# Autodesk Inventor assembly: NoSpace2.0
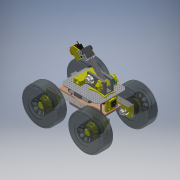
[picture p0: Inventor's stored thumbnail of the model, 180x180]
Saved by Autodesk Inventor 2019.1 (Build 231200000, 200)
## iProperties
Created: 2018-10-15
Part Number: NoSpace2.0
Material: Типовые
Document SubType Name: Assembly
Designer: Олег
Author: Олег
## Documents named in this file (34)
- C:\Users\Олег\OneDrive\Общая\NoSpace 2.0\NoSpace2.0.iam
- C:\Users\Олег\OneDrive\Общая\NoSpace 2.0\Основная пластина платформы.ipt
- C:\Users\Олег\OneDrive\Общая\NoSpace 2.0\Линейка.ipt
- C:\Users\Олег\OneDrive\Общая\NoSpace 2.0\Мотор-колесо\Мотор-колесо.iam
- C:\Users\Олег\OneDrive\Общая\NoSpace 2.0\Стойка между первым и вторым этажом.ipt
- C:\Users\Олег\OneDrive\Общая\NoSpace 2.0\Перфорированная пластина второго этажа.ipt
- C:\Users\Олег\OneDrive\Общая\NoSpace 2.0\Манипулятор\Поворотный узел манипулятора\Поворотный узел манипулятора.iam
- C:\Users\Олег\OneDrive\Общая\NoSpace 2.0\Крепление платы раздачи питания.ipt
- C:\Users\Олег\OneDrive\Общая\NoSpace 2.0\Держатель драйвера.ipt
- C:\Users\Олег\OneDrive\Общая\NoSpace 2.0\Малина.ipt
- C:\Users\Олег\OneDrive\Общая\NoSpace 2.0\стойка для платы 10мм.ipt
- C:\Users\Олег\OneDrive\Общая\NoSpace 2.0\bullet корпус.ipt
- C:\Users\Олег\OneDrive\Общая\NoSpace 2.0\bullet крышка.ipt
- C:\Users\Олег\OneDrive\Общая\NoSpace 2.0\Крепление АКБ.ipt
- C:\Users\Олег\OneDrive\Общая\NoSpace 2.0\Камера\Камера raspberry pi.ipt
- C:\Users\Олег\OneDrive\Общая\NoSpace 2.0\Камера\Основа камеры.ipt
- C:\Users\Олег\OneDrive\Общая\NoSpace 2.0\Камера\Поворотная платформа камеры.ipt
- C:\Users\Олег\OneDrive\Общая\NoSpace 2.0\Камера\Проставка между камерой и поворотной платформой.ipt
- C:\Users\Олег\OneDrive\Общая\NoSpace 2.0\Камера\Фиксатор подшипнкиа камеры.ipt
- C:\Users\Олег\OneDrive\Общая\NoSpace 2.0\Камера\Servo-MG90S.ipt
- C:\Users\Олег\OneDrive\Общая\NoSpace 2.0\Камера\Подшипник 3x10x4.ipt
- C:\Users\Олег\OneDrive\Общая\NoSpace 2.0\Манипулятор\Блок подъёма первога звена\Основная часть подъемного механизма первого звена.iam
- C:\Users\Олег\OneDrive\Общая\NoSpace 2.0\Манипулятор\Блок подъёма первога звена\Ось подъёмного блока первого звена.ipt
- C:\Users\Олег\OneDrive\Общая\NoSpace 2.0\Манипулятор\Блок подъёма первога звена\Узел потенциометра.iam
- C:\Users\Олег\OneDrive\Общая\NoSpace 2.0\Манипулятор\Блок подъёма первога звена\Шкив.iam
- C:\Users\Олег\OneDrive\Общая\NoSpace 2.0\Мотор-колесо\Мотор\Мотор.iam
- C:\Users\Олег\OneDrive\Общая\NoSpace 2.0\Манипулятор\Блок подъёма первога звена\Съёмное крепление мотора 37мм.ipt
- C:\Users\Олег\OneDrive\Общая\NoSpace 2.0\Манипулятор\Блок подъёма первога звена\Переходник от первого звена к оси.ipt
- C:\Users\Олег\OneDrive\Общая\NoSpace 2.0\Манипулятор\Блок подъёма первога звена\Шкив.ipt
- C:\Users\Олег\OneDrive\Общая\NoSpace 2.0\Манипулятор\Удлинение звена.ipt
- C:\Users\Олег\OneDrive\Общая\NoSpace 2.0\Манипулятор\Servoarm 1 RDS3115mg.ipt
- C:\Users\Олег\OneDrive\Общая\NoSpace 2.0\Манипулятор\RDS3115 MG.ipt
- C:\Users\Олег\OneDrive\Общая\NoSpace 2.0\Манипулятор\Поворотный узел схвата\Поворотный узел схвата.iam
- C:\Users\Олег\OneDrive\Общая\NoSpace 2.0\Манипулятор\Крепление схвата.ipt
## Components (47 placed, 33 different names)
1. Основная пластина платформы:1 — Совмещение:1, Совмещение:2, Совмещение:3, Совмещение:4, Совмещение:5, Совмещение:6, Совмещение:19, Совмещение:20, Совмещение:21, Совмещение:22, Совмещение:23, Совмещение:24, Совмещение:25, Совмещение:26, Совмещение:33, Совмещение:34, Совмещение:35, Совмещение:36, Совмещение:37, Совмещение:38, Совмещение:39, Заподлицо:1, Совмещение:41, Совмещение:42, Совмещение:43, Совмещение:44, Совмещение:45, Совмещение:46, Совмещение:48
2. Линейка:1 — Совмещение:4, Совмещение:5, Совмещение:6, Совмещение:13, Совмещение:14, Совмещение:15, Совмещение:16, Совмещение:17, Совмещение:18
3. Линейка:2 — Совмещение:1, Совмещение:2, Совмещение:3, Совмещение:7, Совмещение:8, Совмещение:9, Совмещение:10, Совмещение:11, Совмещение:12
4. Мотор-колесо:1 [sub-assembly] — Совмещение:10, Совмещение:11, Совмещение:12
5. Мотор-колесо:2 [sub-assembly] — Совмещение:13, Совмещение:14, Совмещение:15
6. Мотор-колесо:3 [sub-assembly] — Совмещение:16, Совмещение:17, Совмещение:18
7. Мотор-колесо:4 [sub-assembly] — Совмещение:7, Совмещение:8, Совмещение:9
8. Стойка между первым и вторым этажом:1 — Совмещение:25, Совмещение:26, Совмещение:27
9. Стойка между первым и вторым этажом:2 — Совмещение:23, Совмещение:24, Совмещение:28, Совмещение:29
10. Стойка между первым и вторым этажом:3 — Совмещение:21, Совмещение:22
11. Стойка между первым и вторым этажом:4 — Совмещение:19, Совмещение:20
12. Перфорированная пластина второго этажа:1 — Совмещение:27, Совмещение:28, Совмещение:29, Совмещение:30, Совмещение:31, Совмещение:32, Совмещение:52, Совмещение:53, Совмещение:54, Совмещение:56, Совмещение:57, Совмещение:58, Совмещение:62, Угол:1, Совмещение:63, Совмещение:64
13. Поворотный узел манипулятора:1 [sub-assembly] — Совмещение:30, Совмещение:31, Совмещение:32, Совмещение:77, Совмещение:78
14. Крепление платы раздачи питания:1 — Совмещение:33, Совмещение:34, Совмещение:35
15. Держатель драйвера:1 — Совмещение:36, Совмещение:37, Совмещение:38, Совмещение:40
16. Малина:1 — Совмещение:39, Совмещение:40, Заподлицо:1, Совмещение:47
17. стойка для платы 10мм:1 — Совмещение:41, Совмещение:42
18. стойка для платы 10мм:2 — Совмещение:44, Совмещение:47
19. стойка для платы 10мм:3 — Совмещение:43, Совмещение:48
20. стойка для платы 10мм:4 — Совмещение:45, Совмещение:46
21. bullet корпус:1 — Заподлицо:2, Заподлицо:3, Совмещение:55, Совмещение:56, Совмещение:57, Совмещение:58
22. bullet крышка:1 — Заподлицо:2, Заподлицо:3, Совмещение:55
23. Крепление АКБ:1 — Совмещение:49, Совмещение:50, Совмещение:51, Совмещение:52, Совмещение:54
24. Крепление АКБ:2 — Совмещение:49, Совмещение:50, Совмещение:51, Совмещение:53
25. Камера raspberry pi:1 — Совмещение:74, Совмещение:75, Совмещение:76
26. Основа камеры:1 — Совмещение:59, Совмещение:60, Совмещение:61, Совмещение:62, Угол:1, Совмещение:63, Совмещение:64, Совмещение:72, Совмещение:73
27. Поворотная платформа камеры:1 — Совмещение:67, Совмещение:68, Совмещение:69, Совмещение:70, Заподлицо:4, Заподлицо:5, Совмещение:72
28. Проставка между камерой и поворотной платформой:1 — Совмещение:70, Заподлицо:4, Заподлицо:5, Совмещение:74, Совмещение:75, Совмещение:76
29. Фиксатор подшипнкиа камеры:1 — Совмещение:59, Совмещение:60, Совмещение:61, Совмещение:65, Совмещение:66
30. Servo-MG90S:1 — Совмещение:67, Совмещение:68, Совмещение:69, Совмещение:73
31. Подшипник 3x10x4:1 — Совмещение:65, Совмещение:66
32. Основная часть подъемного механизма первого звена:1 [sub-assembly] — Совмещение:77, Совмещение:78, Совмещение:79, Совмещение:81, Заподлицо:6, Совмещение:86, Совмещение:87, Совмещение:88, Совмещение:89, Совмещение:94, Совмещение:110
33. Ось подъёмного блока первого звена:1 — Совмещение:81, Заподлицо:6, Совмещение:85, Совмещение:90, Заподлицо:7
34. Узел потенциометра:1 [sub-assembly] — Совмещение:87, Совмещение:88, Совмещение:89
35. Шкив:1 [sub-assembly] — Совмещение:90, Заподлицо:7, Угол:3
36. Мотор:1 [sub-assembly] — Совмещение:83, Совмещение:95, Совмещение:96, Совмещение:101, Заподлицо:8
37. Съёмное крепление мотора 37мм:1 — Совмещение:79, Совмещение:83, Совмещение:94, Совмещение:95, Совмещение:101, Совмещение:110
38. Переходник от первого звена к оси:1 — Совмещение:85, Совмещение:86, Угол:3, Совмещение:102, Совмещение:103, Совмещение:104, Совмещение:105, Совмещение:106, Совмещение:107, Совмещение:108, Совмещение:109, Угол:4
39. Синхронный шкив2:1 — Совмещение:96, Заподлицо:8
40. Удлинение звена:1 — Совмещение:104, Совмещение:105, Совмещение:114, Совмещение:115
41. Удлинение звена:2 — Совмещение:106, Совмещение:107
42. Удлинение звена:3 — Совмещение:102, Совмещение:103
43. Удлинение звена:4 — Совмещение:108, Совмещение:109
44. Servoarm 1 RDS3115mg:1 — Совмещение:111, Совмещение:112, Совмещение:113, Совмещение:114, Совмещение:115, Угол:4
45. RDS3115 MG:1 — Совмещение:111, Совмещение:112, Совмещение:113, Совмещение:117, Совмещение:120
46. Поворотный узел схвата:1 [sub-assembly] — Совмещение:117, Совмещение:118, Совмещение:119, Совмещение:120
47. Крепление схвата:1 — Совмещение:118, Совмещение:119
## Relationships (119: Mate 108, Flush 8, Angle 3)
- Совмещение:1 [Mate]: Основная пластина платформы:1 ↔ Линейка:2
- Совмещение:2 [Mate]: Основная пластина платформы:1 ↔ Линейка:2
- Совмещение:3 [Mate]: Основная пластина платформы:1 ↔ Линейка:2
- Совмещение:4 [Mate]: Основная пластина платформы:1 ↔ Линейка:1
- Совмещение:5 [Mate]: Основная пластина платформы:1 ↔ Линейка:1
- Совмещение:6 [Mate]: Основная пластина платформы:1 ↔ Линейка:1
- Совмещение:7 [Mate]: Линейка:2 ↔ Мотор-колесо:4
- Совмещение:8 [Mate]: Линейка:2 ↔ Мотор-колесо:4
- Совмещение:9 [Mate]: Линейка:2 ↔ Мотор-колесо:4
- Совмещение:10 [Mate]: Линейка:2 ↔ Мотор-колесо:1
- Совмещение:11 [Mate]: Линейка:2 ↔ Мотор-колесо:1
- Совмещение:12 [Mate]: Линейка:2 ↔ Мотор-колесо:1
- Совмещение:13 [Mate]: Линейка:1 ↔ Мотор-колесо:2
- Совмещение:14 [Mate]: Линейка:1 ↔ Мотор-колесо:2
- Совмещение:15 [Mate]: Линейка:1 ↔ Мотор-колесо:2
- Совмещение:16 [Mate]: Линейка:1 ↔ Мотор-колесо:3
- Совмещение:17 [Mate]: Линейка:1 ↔ Мотор-колесо:3
- Совмещение:18 [Mate]: Линейка:1 ↔ Мотор-колесо:3
- Совмещение:19 [Mate]: Основная пластина платформы:1 ↔ Стойка между первым и вторым этажом:4
- Совмещение:20 [Mate]: Основная пластина платформы:1 ↔ Стойка между первым и вторым этажом:4
- Совмещение:21 [Mate]: Основная пластина платформы:1 ↔ Стойка между первым и вторым этажом:3
- Совмещение:22 [Mate]: Основная пластина платформы:1 ↔ Стойка между первым и вторым этажом:3
- Совмещение:23 [Mate]: Основная пластина платформы:1 ↔ Стойка между первым и вторым этажом:2
- Совмещение:24 [Mate]: Основная пластина платформы:1 ↔ Стойка между первым и вторым этажом:2
- Совмещение:25 [Mate]: Основная пластина платформы:1 ↔ Стойка между первым и вторым этажом:1
- Совмещение:26 [Mate]: Основная пластина платформы:1 ↔ Стойка между первым и вторым этажом:1
- Совмещение:27 [Mate]: Стойка между первым и вторым этажом:1 ↔ Перфорированная пластина второго этажа:1
- Совмещение:28 [Mate]: Стойка между первым и вторым этажом:2 ↔ Перфорированная пластина второго этажа:1
- Совмещение:29 [Mate]: Стойка между первым и вторым этажом:2 ↔ Перфорированная пластина второго этажа:1
- Совмещение:30 [Mate]: Перфорированная пластина второго этажа:1 ↔ Поворотный узел манипулятора:1
- Совмещение:31 [Mate]: Перфорированная пластина второго этажа:1 ↔ Поворотный узел манипулятора:1
- Совмещение:32 [Mate]: Перфорированная пластина второго этажа:1 ↔ Поворотный узел манипулятора:1
- Совмещение:33 [Mate]: Основная пластина платформы:1 ↔ Крепление платы раздачи питания:1
- Совмещение:34 [Mate]: Основная пластина платформы:1 ↔ Крепление платы раздачи питания:1
- Совмещение:35 [Mate]: Основная пластина платформы:1 ↔ Крепление платы раздачи питания:1
- Совмещение:36 [Mate]: Основная пластина платформы:1 ↔ Держатель драйвера:1
- Совмещение:37 [Mate]: Основная пластина платформы:1 ↔ Держатель драйвера:1
- Совмещение:38 [Mate]: Основная пластина платформы:1 ↔ Держатель драйвера:1
- Совмещение:39 [Mate] (10 mm): Основная пластина платформы:1 ↔ Малина:1
- Совмещение:40 [Mate]: Держатель драйвера:1 ↔ Малина:1
- Заподлицо:1 [Flush] (3 mm): Основная пластина платформы:1 ↔ Малина:1
- Совмещение:41 [Mate]: Основная пластина платформы:1 ↔ стойка для платы 10мм:1
- Совмещение:42 [Mate]: Основная пластина платформы:1 ↔ стойка для платы 10мм:1
- Совмещение:43 [Mate]: Основная пластина платформы:1 ↔ стойка для платы 10мм:3
- Совмещение:44 [Mate]: Основная пластина платформы:1 ↔ стойка для платы 10мм:2
- Совмещение:45 [Mate]: Основная пластина платформы:1 ↔ стойка для платы 10мм:4
- Совмещение:46 [Mate]: Основная пластина платформы:1 ↔ стойка для платы 10мм:4
- Совмещение:47 [Mate]: Малина:1 ↔ стойка для платы 10мм:2
- Совмещение:48 [Mate]: Основная пластина платформы:1 ↔ стойка для платы 10мм:3
- Совмещение:49 [Mate]: Крепление АКБ:1 ↔ Крепление АКБ:2
- Совмещение:50 [Mate]: Крепление АКБ:1 ↔ Крепление АКБ:2
- Совмещение:51 [Mate]: Крепление АКБ:1 ↔ Крепление АКБ:2
- Совмещение:52 [Mate]: Перфорированная пластина второго этажа:1 ↔ Крепление АКБ:1
- Совмещение:53 [Mate]: Перфорированная пластина второго этажа:1 ↔ Крепление АКБ:2
- Совмещение:54 [Mate]: Перфорированная пластина второго этажа:1 ↔ Крепление АКБ:1
- Заподлицо:2 [Flush]: bullet корпус:1 ↔ bullet крышка:1
- Заподлицо:3 [Flush]: bullet корпус:1 ↔ bullet крышка:1
- Совмещение:55 [Mate]: bullet корпус:1 ↔ bullet крышка:1
- Совмещение:56 [Mate]: Перфорированная пластина второго этажа:1 ↔ bullet корпус:1
- Совмещение:57 [Mate]: Перфорированная пластина второго этажа:1 ↔ bullet корпус:1
- Совмещение:58 [Mate]: Перфорированная пластина второго этажа:1 ↔ bullet корпус:1
- Совмещение:59 [Mate]: Основа камеры:1 ↔ Фиксатор подшипнкиа камеры:1
- Совмещение:60 [Mate]: Основа камеры:1 ↔ Фиксатор подшипнкиа камеры:1
- Совмещение:61 [Mate]: Основа камеры:1 ↔ Фиксатор подшипнкиа камеры:1
- Совмещение:62 [Mate]: Перфорированная пластина второго этажа:1 ↔ Основа камеры:1
- Угол:1 [Angle] (0 deg): Перфорированная пластина второго этажа:1 ↔ Основа камеры:1
- Совмещение:63 [Mate]: Перфорированная пластина второго этажа:1 ↔ Основа камеры:1
- Совмещение:64 [Mate]: Перфорированная пластина второго этажа:1 ↔ Основа камеры:1
- Совмещение:65 [Mate]: Фиксатор подшипнкиа камеры:1 ↔ Подшипник 3x10x4:1
- Совмещение:66 [Mate] (0.5 mm): Фиксатор подшипнкиа камеры:1 ↔ Подшипник 3x10x4:1
- Совмещение:67 [Mate]: Поворотная платформа камеры:1 ↔ Servo-MG90S:1
- Совмещение:68 [Mate]: Поворотная платформа камеры:1 ↔ Servo-MG90S:1
- Совмещение:69 [Mate]: Поворотная платформа камеры:1 ↔ Servo-MG90S:1
- Совмещение:70 [Mate]: Поворотная платформа камеры:1 ↔ Проставка между камерой и поворотной платформой:1
- Заподлицо:4 [Flush]: Поворотная платформа камеры:1 ↔ Проставка между камерой и поворотной платформой:1
- Заподлицо:5 [Flush]: Поворотная платформа камеры:1 ↔ Проставка между камерой и поворотной платформой:1
- Совмещение:72 [Mate] (1 mm): Основа камеры:1 ↔ Поворотная платформа камеры:1
- Совмещение:73 [Mate]: Основа камеры:1 ↔ Servo-MG90S:1
- Совмещение:74 [Mate]: Камера raspberry pi:1 ↔ Проставка между камерой и поворотной платформой:1
- Совмещение:75 [Mate]: Камера raspberry pi:1 ↔ Проставка между камерой и поворотной платформой:1
- Совмещение:76 [Mate]: Камера raspberry pi:1 ↔ Проставка между камерой и поворотной платформой:1
- Совмещение:77 [Mate]: Поворотный узел манипулятора:1 ↔ Основная часть подъемного механизма первого звена:1
- Совмещение:78 [Mate]: Поворотный узел манипулятора:1 ↔ Основная часть подъемного механизма первого звена:1
- Совмещение:79 [Mate]: Основная часть подъемного механизма первого звена:1 ↔ Съёмное крепление мотора 37мм:1
- Совмещение:81 [Mate]: Основная часть подъемного механизма первого звена:1 ↔ Ось подъёмного блока первого звена:1
- Заподлицо:6 [Flush]: Основная часть подъемного механизма первого звена:1 ↔ Ось подъёмного блока первого звена:1
- Совмещение:83 [Mate]: Мотор:1 ↔ Съёмное крепление мотора 37мм:1
- Совмещение:85 [Mate]: Ось подъёмного блока первого звена:1 ↔ Переходник от первого звена к оси:1
- Совмещение:86 [Mate]: Основная часть подъемного механизма первого звена:1 ↔ Переходник от первого звена к оси:1
- Совмещение:87 [Mate]: Основная часть подъемного механизма первого звена:1 ↔ Узел потенциометра:1
- Совмещение:88 [Mate]: Основная часть подъемного механизма первого звена:1 ↔ Узел потенциометра:1
- Совмещение:89 [Mate]: Основная часть подъемного механизма первого звена:1 ↔ Узел потенциометра:1
- Совмещение:90 [Mate]: Ось подъёмного блока первого звена:1 ↔ Шкив:1
- Заподлицо:7 [Flush] (2 mm): Ось подъёмного блока первого звена:1 ↔ Шкив:1
- Угол:3 [Angle] (0 deg): Шкив:1 ↔ Переходник от первого звена к оси:1
- Совмещение:94 [Mate]: Основная часть подъемного механизма первого звена:1 ↔ Съёмное крепление мотора 37мм:1
- Совмещение:95 [Mate]: Мотор:1 ↔ Съёмное крепление мотора 37мм:1
- Совмещение:96 [Mate]: Мотор:1 ↔ Синхронный шкив2:1
- Совмещение:101 [Mate]: Мотор:1 ↔ Съёмное крепление мотора 37мм:1
- Совмещение:102 [Mate]: Переходник от первого звена к оси:1 ↔ Удлинение звена:3
- Совмещение:103 [Mate]: Переходник от первого звена к оси:1 ↔ Удлинение звена:3
- Совмещение:104 [Mate]: Переходник от первого звена к оси:1 ↔ Удлинение звена:1
- Совмещение:105 [Mate]: Переходник от первого звена к оси:1 ↔ Удлинение звена:1
- Совмещение:106 [Mate]: Переходник от первого звена к оси:1 ↔ Удлинение звена:2
- Совмещение:107 [Mate]: Переходник от первого звена к оси:1 ↔ Удлинение звена:2
- Совмещение:108 [Mate]: Переходник от первого звена к оси:1 ↔ Удлинение звена:4
- Совмещение:109 [Mate]: Переходник от первого звена к оси:1 ↔ Удлинение звена:4
- Совмещение:110 [Mate] (7.68 mm): Основная часть подъемного механизма первого звена:1 ↔ Съёмное крепление мотора 37мм:1
- Заподлицо:8 [Flush] (4 mm): Мотор:1 ↔ Синхронный шкив2:1
- Совмещение:111 [Mate]: Servoarm 1 RDS3115mg:1 ↔ RDS3115 MG:1
- Совмещение:112 [Mate]: Servoarm 1 RDS3115mg:1 ↔ RDS3115 MG:1
- Совмещение:113 [Mate]: Servoarm 1 RDS3115mg:1 ↔ RDS3115 MG:1
- Совмещение:114 [Mate]: Удлинение звена:1 ↔ Servoarm 1 RDS3115mg:1
- Совмещение:115 [Mate]: Удлинение звена:1 ↔ Servoarm 1 RDS3115mg:1
- Угол:4 [Angle] (0 deg): Переходник от первого звена к оси:1 ↔ Servoarm 1 RDS3115mg:1
- Совмещение:117 [Mate]: RDS3115 MG:1 ↔ Поворотный узел схвата:1
- Совмещение:118 [Mate]: Поворотный узел схвата:1 ↔ Крепление схвата:1
- Совмещение:119 [Mate]: Поворотный узел схвата:1 ↔ Крепление схвата:1
- Совмещение:120 [Mate]: RDS3115 MG:1 ↔ Поворотный узел схвата:1
